# Autodesk Inventor assembly: Assembly_Linear_MGN8_Noncaptive
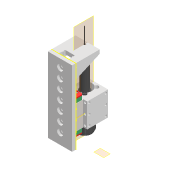
[picture p0: Inventor's stored thumbnail of the model, 180x180]
Saved by Autodesk Inventor 2022 (Build 260153000, 153)
## iProperties
Created: 2022-12-17
Part Number: Assembly_Linear_MGN8_Noncaptive
Document SubType Name: Assembly
Designer: diederichbenedict
Author: diederichbenedict
## Documents named in this file (6)
- C:\Users\diederichbenedict\Dropbox\Dokumente\Promotion\PROJECTS\openUC2-CAD\INVENTOR\Assembly_Linear_MGN8_Noncaptive.iam
- C:\Users\diederichbenedict\Dropbox\Dokumente\Promotion\PROJECTS\openUC2-CAD\INVENTOR\00_MGN12H, LINEAR GUIDE BLOCK.ipt
- C:\Users\diederichbenedict\Dropbox\Dokumente\Promotion\PROJECTS\openUC2-CAD\INVENTOR\00_MGN12H, LINEAR Rail.ipt
- C:\Users\diederichbenedict\Dropbox\Dokumente\Promotion\PROJECTS\openUC2-CAD\INVENTOR\00_Joy-IT-B20SHD4353_NEMA8_captive.ipt
- C:\Users\diederichbenedict\Dropbox\Dokumente\Promotion\PROJECTS\openUC2-CAD\INVENTOR\30_Linear_Captive_Nema8_Guidemount.ipt
- C:\Users\diederichbenedict\Dropbox\Dokumente\Promotion\PROJECTS\openUC2-CAD\INVENTOR\30_Linear_Captive_Nema8_Base.ipt
## Components (5 placed, 5 different names)
1. 00_MGN12H, LINEAR GUIDE BLOCK:1 — Fluchtend:1, Passend:1, Passend:2, Fluchtend:3, Fluchtend:4, Fluchtend:5
2. 00_MGN12H, LINEAR Rail:1 — Fluchtend:1, Passend:1, Fluchtend:2, Fluchtend:7, Fluchtend:8
3. 00_Joy-IT-B20SHD4353_NEMA8_captive:1 — Fluchtend:2, Passend:2, Fluchtend:3, Fluchtend:6
4. 30_Linear_Captive_Nema8_Guidemount:1 — Fluchtend:4, Fluchtend:5, Fluchtend:6
5. 30_Linear_Captive_Nema8_Base:1 — Fluchtend:7, Fluchtend:8
## Relationships (10: Flush 8, Mate 2)
- Fluchtend:1 [Flush]: 00_MGN12H, LINEAR GUIDE BLOCK:1 ↔ 00_MGN12H, LINEAR Rail:1
- Passend:1 [Mate]: 00_MGN12H, LINEAR GUIDE BLOCK:1 ↔ 00_MGN12H, LINEAR Rail:1
- Fluchtend:2 [Flush]: 00_MGN12H, LINEAR Rail:1 ↔ 00_Joy-IT-B20SHD4353_NEMA8_captive:1
- Passend:2 [Mate] (5 mm): 00_MGN12H, LINEAR GUIDE BLOCK:1 ↔ 00_Joy-IT-B20SHD4353_NEMA8_captive:1
- Fluchtend:3 [Flush] (2 mm): 00_MGN12H, LINEAR GUIDE BLOCK:1 ↔ 00_Joy-IT-B20SHD4353_NEMA8_captive:1
- Fluchtend:4 [Flush] (3 mm): 00_MGN12H, LINEAR GUIDE BLOCK:1 ↔ 30_Linear_Captive_Nema8_Guidemount:1
- Fluchtend:5 [Flush]: 00_MGN12H, LINEAR GUIDE BLOCK:1 ↔ 30_Linear_Captive_Nema8_Guidemount:1
- Fluchtend:6 [Flush]: 00_Joy-IT-B20SHD4353_NEMA8_captive:1 ↔ 30_Linear_Captive_Nema8_Guidemount:1
- Fluchtend:7 [Flush]: 00_MGN12H, LINEAR Rail:1 ↔ 30_Linear_Captive_Nema8_Base:1
- Fluchtend:8 [Flush]: 00_MGN12H, LINEAR Rail:1 ↔ 30_Linear_Captive_Nema8_Base:1
